# Autodesk Inventor assembly: shin_assembly
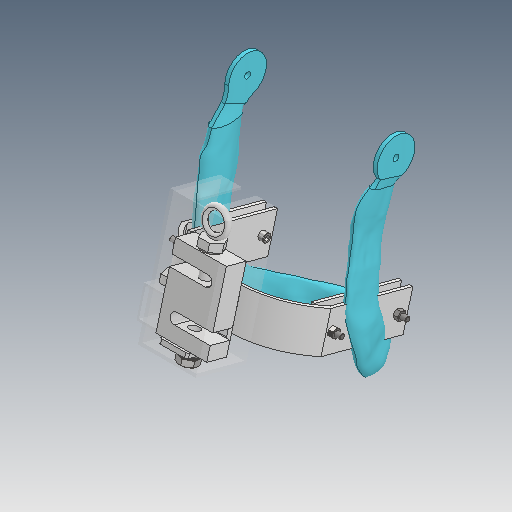
[picture p0: Inventor's stored thumbnail of the model, 512x512]
Saved by Autodesk Inventor 2025.2 (Build 292293000, 293)
## iProperties
Created: 2025-02-17
Part Number: shin_assembly
Document SubType Name: Assembly
Designer: email
Author: email
## Documents named in this file (3)
- C:\Users\email\Desktop\Projects\Capstone\4TB6\CAD_Model\thigh_mount_2\shin_assembly.iam
- C:\Users\email\Desktop\Projects\Capstone\4TB6\CAD_Model\thigh_mount_2\shin.ipt
- C:\Users\email\Desktop\Projects\Capstone\4TB6\CAD_Model\thigh_mount_2\shin_bracket_assem.iam
## Components (2 placed, 2 different names)
1. shin:1 — Flush:2, Mate:1, Angle:1, Mate:2, Mate:3
2. shin_bracket_assem:1 [sub-assembly] — Flush:2, Mate:1, Angle:1, Mate:2, Mate:3
## Relationships (5: Mate 3, Flush 1, Angle 1)
- Flush:2 (-120 mm): shin:1 ↔ shin_bracket_assem:1
- Mate:1 (60 mm): shin:1 ↔ shin_bracket_assem:1
- Angle:1 (15 deg): shin:1 ↔ shin_bracket_assem:1
- Mate:2: shin:1 ↔ shin_bracket_assem:1
- Mate:3 (120 mm): shin:1 ↔ shin_bracket_assem:1
